# Autodesk Inventor assembly: assembly
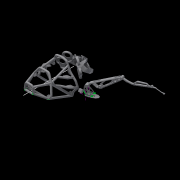
[picture p0: Inventor's stored thumbnail of the model, 180x180]
Saved by Autodesk Inventor 2020 (Build 240168000, 168)
## iProperties
Created: 2020-03-24
Part Number: assembly
Document SubType Name: Assembly
Designer: valer
Author: valer
## Documents named in this file (8)
- C:\Users\valer\Desktop\drummingrobot\src\Robot.iam
- C:\Users\valer\Desktop\drummingrobot\src\Chest.ipt
- C:\Users\valer\Desktop\drummingrobot\src\HeadScaled.ipt
- C:\Users\valer\Desktop\drummingrobot\src\UpperArmServoDynamixelXM430-W350-T.ipt
- C:\Users\valer\Desktop\drummingrobot\src\Forearm.ipt
- C:\Users\valer\Desktop\drummingrobot\src\UpperArmGenerative v6.ipt
- C:\Users\valer\Desktop\drummingrobot\src\UpperArmBracket.ipt
- C:\Users\valer\Desktop\drummingrobot\src\UpperArmMount.ipt
## Components (8 placed, 7 different names)
1. Chest:1 — Angle:1
2. HeadScaled:1
3. UpperArmServoDynamixelXM430-W350-T:1 — Angle:1
4. Forearm:1 — Mate:1, Flush:1
5. UpperArm:1 — Mate:1, Flush:1, Mate:2, Mate:3, Mate:4, Mate:5
6. UpperArmBracket:1 — Mate:2, Mate:3, Mate:6, Mate:8, Mate:9
7. UpperArmMount:1 — Mate:6, Mate:7, Mate:8, Mate:9
8. UpperArmBracket:2 — Mate:4, Mate:5, Mate:7
## Relationships (11: Mate 9, Angle 1, Flush 1)
- Angle:1 (0 deg): Chest:1 ↔ UpperArmServoDynamixelXM430-W350-T:1
- Mate:1: Forearm:1 ↔ UpperArm:1
- Flush:1 (12.7 mm): Forearm:1 ↔ UpperArm:1
- Mate:2: UpperArm:1 ↔ UpperArmBracket:1
- Mate:3: UpperArm:1 ↔ UpperArmBracket:1
- Mate:4: UpperArm:1 ↔ UpperArmBracket:2
- Mate:5: UpperArm:1 ↔ UpperArmBracket:2
- Mate:6: UpperArmBracket:1 ↔ UpperArmMount:1
- Mate:7: UpperArmMount:1 ↔ UpperArmBracket:2
- Mate:8: UpperArmBracket:1 ↔ UpperArmMount:1
- Mate:9 (12.7 mm): UpperArmBracket:1 ↔ UpperArmMount:1
